# Autodesk Inventor assembly: 2sr_ass_1
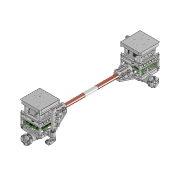
[picture p0: Inventor's stored thumbnail of the model, 180x180]
Saved by Autodesk Inventor 2020 (Build 240168000, 168)
## iProperties
Created: 2022-07-09
Part Number: 2sr_ass_1
Document SubType Name: Assembly
Designer: Shuang Peng
Author: Shuang Peng
## Documents named in this file (5)
- D:\projects-3\soft module robot\hardware\diff module 3\2sr_ass_1.iam
- D:\projects-3\soft module robot\hardware\diff module 3\base_ass_3.iam
- D:\projects-3\soft module robot\hardware\diff module 3\bridge_1.ipt
- D:\projects-3\soft module robot\hardware\diff module 3\coil_in.ipt
- D:\projects-3\soft module robot\hardware\diff module 3\bridge_inner_s1.ipt
## Components (6 placed, 4 different names)
1. base_ass_3:1 [sub-assembly] — Insert:1, Flush:1
2. base_ass_3:2 [sub-assembly] — Insert:2, Flush:1
3. bridge_1:1 — Insert:1, Insert:2, Insert:3, Insert:4
4. coil_in:1 — Insert:3
5. coil_in:2 — Insert:4, Insert:5
6. bridge_inner_s1:1 — Insert:5
## Relationships (6: Insert 5, Flush 1)
- Insert:1: base_ass_3:1 ↔ bridge_1:1
- Insert:2: base_ass_3:2 ↔ bridge_1:1
- Flush:1: base_ass_3:1 ↔ base_ass_3:2
- Insert:3 (15 mm): bridge_1:1 ↔ coil_in:1
- Insert:4 (15 mm): bridge_1:1 ↔ coil_in:2
- Insert:5: coil_in:2 ↔ bridge_inner_s1:1
